# Autodesk Inventor assembly: structure
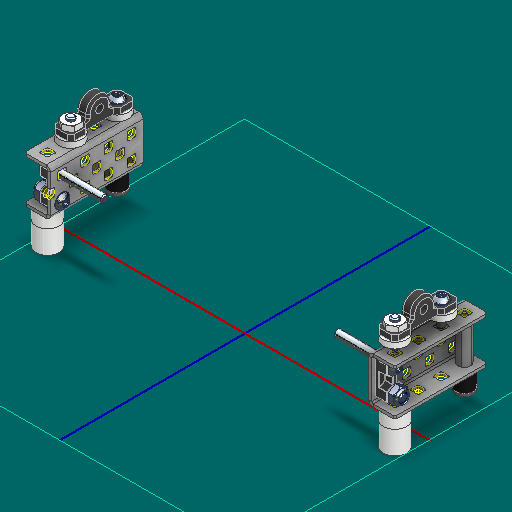
[picture p0: Inventor's stored thumbnail of the model, 512x512]
Saved by Autodesk Inventor 2025 (Build 290162000, 162)
## iProperties
Created: 2024-08-18
Part Number: structure
Document SubType Name: Assembly
Designer: averey
Author: averey
## Documents named in this file (3)
- C:\Users\avere\vex_robotics_high_stakes\hardware\cad\ATLAS\intake\first_stage\structure.iam
- C:\Users\avere\vex_robotics_high_stakes\hardware\cad\ATLAS\intake\first_stage\tower.iam
- C:\Users\avere\vex_robotics_high_stakes\hardware\cad\ATLAS\intake\first_stage\tower_mirrored\tower_mirrored.iam
## Components (2 placed, 2 different names)
1. tower:1 [sub-assembly] — Insert:1, Mate:1, Mate:2, Mate:3
2. tower_mirrored:1 [sub-assembly] — Insert:1, Mate:1
## Relationships (4: Mate 3, Insert 1)
- Insert:1 (174.625 mm): tower:1 ↔ tower_mirrored:1
- Mate:1: tower:1 ↔ tower_mirrored:1
- Mate:2: tower:1
- Mate:3 (95.25 mm): tower:1
